# Autodesk Inventor assembly: model_awds
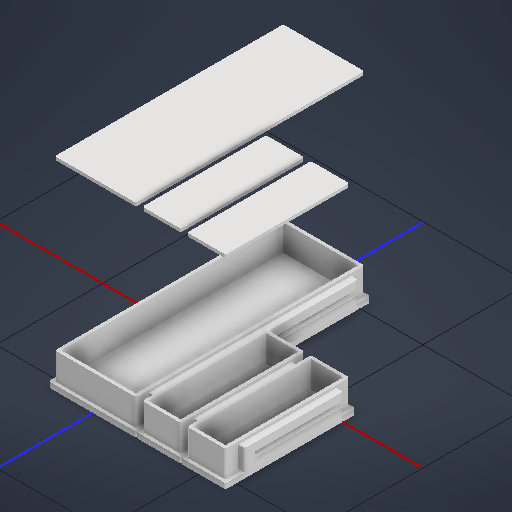
[picture p0: Inventor's stored thumbnail of the model, 512x512]
Saved by Autodesk Inventor 2025.2 (Build 292293000, 293)
## iProperties
Created: 2025-09-05
Part Number: model_awds
Document SubType Name: Assembly
Designer: sam
Author: sam
## Documents named in this file (5)
- G:\projects\primary\auto-water-distribution-system\model\assembly\model_awds.iam
- G:\projects\primary\auto-water-distribution-system\model\assembly\parts\module_command.ipt
- G:\projects\primary\auto-water-distribution-system\model\assembly\parts\module-lid_command.ipt
- G:\projects\primary\auto-water-distribution-system\model\assembly\parts\module_switch.ipt
- G:\projects\primary\auto-water-distribution-system\model\assembly\parts\module-lid_switch.ipt
## Components (6 placed, 4 different names)
1. module_command:1 — Mate:1, Mate:2, Flush:1, Mate:3, Mate:4, Flush:2
2. module-lid_command:1 — Mate:1, Mate:2, Flush:3, Flush:4
3. module_switch:1 — Flush:1, Mate:3, Mate:4, Mate:5, Mate:6, Mate:7, Mate:8
4. module_switch:2 — Flush:2, Mate:5, Mate:6, Mate:9, Mate:10
5. module-lid_switch:1 — Flush:3, Mate:7, Mate:8
6. module-lid_switch:2 — Flush:4, Mate:9, Mate:10
## Relationships (14: Mate 10, Flush 4)
- Mate:1: module_command:1 ↔ module-lid_command:1
- Mate:2: module_command:1 ↔ module-lid_command:1
- Flush:1: module_command:1 ↔ module_switch:1
- Mate:3: module_command:1 ↔ module_switch:1
- Mate:4: module_command:1 ↔ module_switch:1
- Flush:2: module_command:1 ↔ module_switch:2
- Mate:5: module_switch:1 ↔ module_switch:2
- Mate:6: module_switch:1 ↔ module_switch:2
- Flush:3: module-lid_command:1 ↔ module-lid_switch:1
- Flush:4: module-lid_command:1 ↔ module-lid_switch:2
- Mate:7: module_switch:1 ↔ module-lid_switch:1
- Mate:8: module_switch:1 ↔ module-lid_switch:1
- Mate:9: module_switch:2 ↔ module-lid_switch:2
- Mate:10: module_switch:2 ↔ module-lid_switch:2
